# Autodesk Inventor assembly: EL2-A-100
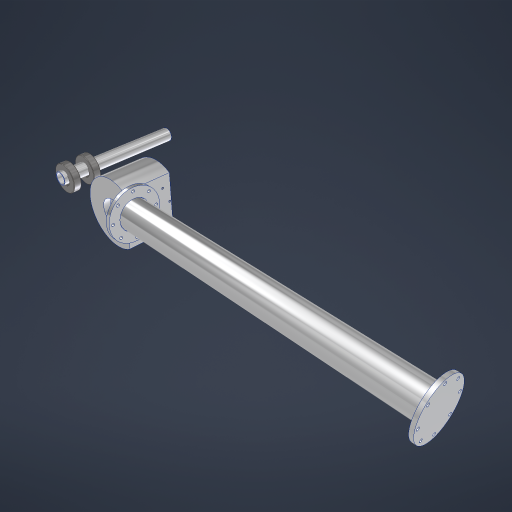
[picture p0: Inventor's stored thumbnail of the model, 512x512]
Saved by Autodesk Inventor 2023.4 (Build 274418000, 418)
## iProperties
Created: 2025-01-11
Part Number: EL2-A-100
Document SubType Name: Assembly
Designer: brand
Author: brand
## Documents named in this file (6)
- C:\Users\brand\OneDrive\Documents\GitHub\robotics 23\2025-ReefScape---CAD\Elevator\EL2\EL2-A-100.iam
- C:\Users\brand\OneDrive\Documents\GitHub\robotics 23\2025-ReefScape---CAD\Elevator\EL2\EL2-C-004.ipt
- C:\Users\brand\OneDrive\Documents\GitHub\robotics 23\2025-ReefScape---CAD\Elevator\EL2\EL2-A-002.ipt
- C:\Users\brand\OneDrive\Documents\GitHub\robotics 23\2025-ReefScape---CAD\Elevator\EL2\EL2-A-003.ipt
- C:\Users\brand\OneDrive\Documents\GitHub\robotics 23\2025-ReefScape---CAD\COMMON PARTS\BEARINGS\0_875_ID_x_1_875_OD_X_0_500_Radial_Bearing_EE11S-2RS.ipt
- C:\Users\brand\OneDrive\Documents\GitHub\robotics 23\2025-ReefScape---CAD\Elevator\EL2\EL2-A-004.ipt
## Components (7 placed, 5 different names)
1. EL2-C-004:1
2. EL2-A-002:1 — Insert:1, Flush:1, Insert:2, Flush:2
3. EL2-A-003:1 — Insert:1, Flush:1
4. EL2-A-003:2 — Insert:2, Flush:2
5. 0_875_ID_x_1_875_OD_X_0_500_Radial_Bearing_EE11S-2RS:1
6. 0_875_ID_x_1_875_OD_X_0_500_Radial_Bearing_EE11S-2RS:2
7. EL2-A-004:1
## Relationships (4: Insert 2, Flush 2)
- Insert:1: EL2-A-002:1 ↔ EL2-A-003:1
- Flush:1: EL2-A-002:1 ↔ EL2-A-003:1
- Insert:2: EL2-A-002:1 ↔ EL2-A-003:2
- Flush:2: EL2-A-002:1 ↔ EL2-A-003:2
